# Autodesk Inventor assembly: AssyClimber
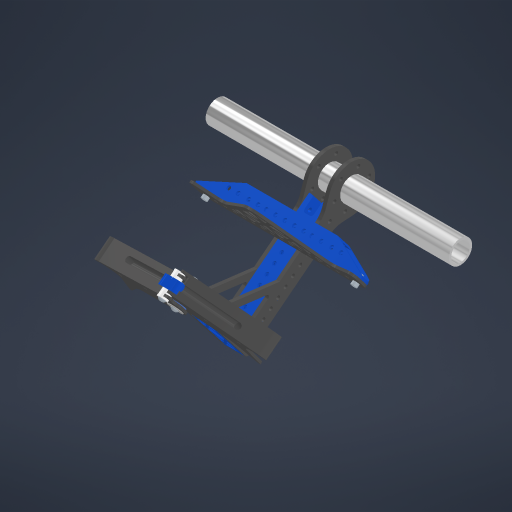
[picture p0: Inventor's stored thumbnail of the model, 512x512]
Saved by Autodesk Inventor 2024.3 (Build 283343000, 343)
## iProperties
Created: 2025-03-19
Part Number: AssyClimber
Document SubType Name: Assembly
Designer: jings
Mass: 1540.49 g
Surface Area: 4241.18 cm^2
Volume: 681.81 cm^3
Author: jings
## Documents named in this file (6)
- C:\Users\jings\OneDrive\Desktop\FRC 5885\2025-Poseidon-Mechanical\climber\AssyClimber.iam
- C:\Users\jings\OneDrive\Desktop\FRC 5885\2025-Poseidon-Mechanical\climber\ClimberBottomBrace.ipt
- C:\Users\jings\OneDrive\Desktop\FRC 5885\2025-Poseidon-Mechanical\climber\ClimberFrame.ipt
- C:\Users\jings\OneDrive\Desktop\FRC 5885\2025-Poseidon-Mechanical\climber\ClimberHook1.ipt
- C:\Users\jings\OneDrive\Desktop\FRC 5885\2025-Poseidon-Mechanical\climber\ClimberHook2.ipt
- C:\Users\jings\OneDrive\Desktop\FRC 5885\2025-Poseidon-Mechanical\climber\ClimberAxel.ipt
## Components (5 placed, 5 different names)
1. ClimberAxel:1 — Mate:1, Insert:6
2. ClimberBottomBrace:1 — Insert:3, Insert:4
3. ClimberFrame:1 — Insert:1, Insert:2, Insert:3, Insert:4, Insert:6, Tangent:2, Tangent:3
4. ClimberHook1:1 — Insert:1, Tangent:3
5. ClimberHook2:1 — Insert:2, Tangent:2
## Relationships (8: Insert 5, Tangent 2, Mate 1)
- Insert:1: ClimberFrame:1 ↔ ClimberHook1:1
- Insert:2: ClimberFrame:1 ↔ ClimberHook2:1
- Insert:3: ClimberBottomBrace:1 ↔ ClimberFrame:1
- Insert:4: ClimberBottomBrace:1 ↔ ClimberFrame:1
- Insert:6 (-147.6375 mm): ClimberAxel:1 ↔ ClimberFrame:1
- Tangent:2: ClimberFrame:1 ↔ ClimberHook2:1
- Tangent:3: ClimberFrame:1 ↔ ClimberHook1:1
- Mate:1: ClimberAxel:1
